# Autodesk Inventor assembly: stage1-planetary
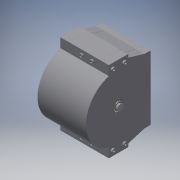
[picture p0: Inventor's stored thumbnail of the model, 180x180]
Saved by Autodesk Inventor 2019 (Build 230136000, 136)
## iProperties
Created: 2019-12-31
Part Number: stage1-planetary
Material: 一般
Document SubType Name: Assembly
Designer: user
Author: user
## Documents named in this file (23)
- D:\大學\大三上\機械設計(宋震國\stage1-planetary.iam
- D:\大學\大三上\機械設計(宋震國\Stage1\Gear_Housing_Bottom.ipt
- D:\大學\大三上\機械設計(宋震國\Stage1\carrier1.ipt
- D:\大學\大三上\機械設計(宋震國\Stage1\planet1.ipt
- D:\大學\大三上\機械設計(宋震國\Stage1\ring1.ipt
- D:\大學\大三上\機械設計(宋震國\Stage1\sun1.ipt
- D:\大學\大三上\機械設計(宋震國\stage1-planetary\機械便覽魔法師\軸5.iam
- D:\大學\大三上\機械設計(宋震國\stage1-planetary\機械便覽魔法師\軸承14.iam
- D:\大學\大三上\機械設計(宋震國\Stage1\planet2.ipt
- D:\大學\大三上\機械設計(宋震國\Stage1\ring2.ipt
- D:\大學\大三上\機械設計(宋震國\Stage1\sun2.ipt
- D:\大學\大三上\機械設計(宋震國\子彧-20200102T093658Z-001\子彧\最後確定\carrier2.ipt
- D:\大學\大三上\機械設計(宋震國\Stage1\Gear_Housing_Input_lid.ipt
- D:\大學\大三上\機械設計(宋震國\Stage1\Gear_Housing_Output_lid.ipt
- D:\大學\大三上\機械設計(宋震國\stage1-planetary\機械便覽魔法師\軸承15.iam
- D:\大學\大三上\機械設計(宋震國\stage1-planetary\機械便覽魔法師\軸承16.iam
- D:\大學\大三上\機械設計(宋震國\stage1-planetary\機械便覽魔法師\軸承17.iam
- D:\大學\大三上\機械設計(宋震國\stage1-planetary\機械便覽魔法師\軸承18.iam
- D:\大學\大三上\機械設計(宋震國\stage1-planetary\機械便覽魔法師\軸6.iam
- D:\大學\大三上\機械設計(宋震國\stage1-planetary\機械便覽魔法師\軸7.iam
- D:\大學\大三上\機械設計(宋震國\Stage1\Gear_Housing_Top2.ipt
- D:\大學\大三上\機械設計(宋震國\Stage1\M4set_screw.ipt
- D:\大學\大三上\機械設計(宋震國\Stage1\M6screw.ipt
## Components (69 placed, 12 different names)
1. Gear_Housing_Bottom:1 — 貼合:92, 貼合:93, 貼合:94, 貼合:95, 貼合:133, 貼合:134, 齊平:38, 貼合:143, 齊平:39, 齊平:41, 貼合:147, 齊平:42, 貼合:148
2. carrier1:1 — 貼合:74, 貼合:75, 貼合:76, 貼合:77, 貼合:78, 貼合:79, 貼合:80, 齊平:15, 齊平:16, 齊平:17, 貼合:176, 貼合:178, 貼合:179, 貼合:180, 貼合:181, 貼合:182, 貼合:183, 貼合:184, 貼合:185, 貼合:186, 貼合:187, 貼合:188, 貼合:189, 貼合:190, 貼合:191, 貼合:192
3. 正齒輪1:6 — 貼合:75, 貼合:84, 插入:2, 貼合:88, 齊平:20
4. 正齒輪2:1 — 貼合:73, 齊平:14, 齊平:21, 貼合:92, 貼合:93
5. 正齒輪1:7 — 貼合:73, 齊平:14, 貼合:74, 旋轉:1, 插入:5, 貼合:175, 貼合:197, 貼合:198
6. 軸:2 [sub-assembly] — 貼合:80, 齊平:17, 貼合:84
7. 正齒輪1:8 — 貼合:76, 貼合:81, 貼合:82, 貼合:87, 齊平:19, 齊平:21
8. 正齒輪1:9 — 貼合:77, 貼合:83, 貼合:85, 齊平:18, 旋轉:1
9. 軸:3 [sub-assembly] — 貼合:78, 齊平:15, 貼合:83, 貼合:86, 插入:4
10. 軸:4 [sub-assembly] — 貼合:79, 貼合:81, 齊平:16, 貼合:82, 插入:3
11. 軸承:1 [sub-assembly] — 貼合:85, 貼合:86, 齊平:18
12. 軸承:3 [sub-assembly] — 插入:3
13. 軸承:4 [sub-assembly] — 貼合:87, 齊平:19
14. 軸承:5 [sub-assembly] — 貼合:88, 齊平:20
15. 軸承:6 [sub-assembly] — 插入:4
16. 軸承:7 [sub-assembly] — 插入:2
17. 軸承:8 [sub-assembly] — 貼合:102, 齊平:28
18. 正齒輪1:11 — 貼合:94, 貼合:95, 貼合:96, 齊平:22, 齊平:36
19. 正齒輪1:12 — 貼合:102, 齊平:28, 貼合:105, 齊平:29, 貼合:106
20. 正齒輪1:13 — 貼合:96, 齊平:22, 貼合:124, 貼合:193, 貼合:194, 貼合:195, 貼合:196
21. 正齒輪1:15 — 貼合:103, 齊平:25, 齊平:32, 貼合:110, 貼合:113, 齊平:36
22. 軸:6 [sub-assembly] — 貼合:113, 貼合:117, 齊平:35, 貼合:119
23. 軸:7 [sub-assembly] — 貼合:116, 齊平:34, 貼合:122, 貼合:123
24. 軸:8 [sub-assembly] — 貼合:106, 貼合:107, 貼合:118, 齊平:33
25. 軸承:9 [sub-assembly] — 貼合:105, 齊平:29, 貼合:107
26. 軸承:12 [sub-assembly] — 齊平:32, 貼合:110, 貼合:119
27. 軸承:13 [sub-assembly] — 貼合:103, 齊平:25
28. 軸承:14 [sub-assembly] — 貼合:120, 貼合:121, 貼合:122
29. carrier2:1 — 貼合:116, 貼合:117, 貼合:118, 齊平:33, 齊平:34, 齊平:35, 貼合:124, 貼合:145, 貼合:199, 貼合:200, 貼合:201, 貼合:202, 貼合:203, 貼合:204
30. 正齒輪1:16 — 貼合:120, 貼合:121, 貼合:123
31. Gear_Housing_Input_lid:1 — 貼合:135, 貼合:136, 貼合:137, 貼合:138, 齊平:38, 貼合:143, 貼合:153, 貼合:160, 貼合:161, 貼合:162, 貼合:163, 貼合:164, 貼合:165, 貼合:166
32. Gear_Housing_Output_lid:1 — 貼合:139, 貼合:140, 貼合:141, 齊平:37, 齊平:39, 貼合:148, 貼合:149, 貼合:167, 貼合:168, 貼合:169, 貼合:170, 貼合:171, 貼合:172, 貼合:173, 貼合:174
33. 軸承:15 [sub-assembly] — 貼合:135, 貼合:136
34. 軸承:16 [sub-assembly] — 貼合:137, 貼合:138, 貼合:142
35. 軸承:17 [sub-assembly] — 貼合:139, 貼合:140
36. 軸承:18 [sub-assembly] — 貼合:141, 齊平:37, 插入:6
37. 軸:11 [sub-assembly] — 貼合:145, 插入:6
38. 軸:12 [sub-assembly] — 插入:5, 貼合:142
39. Gear_Housing_Top2:1 — 貼合:147, 齊平:42, 貼合:149, 貼合:151, 貼合:152, 貼合:154, 貼合:155, 貼合:156, 貼合:157, 貼合:158, 貼合:159
40. M4set_screw:1 — 貼合:179, 貼合:180
41. M6screw:1 — 貼合:151, 貼合:159
42. M4set_screw:2 — 貼合:176, 貼合:182
43. M6screw:2 — 貼合:152, 貼合:158
44. M4set_screw:3 — 貼合:178, 貼合:181
45. M6screw:3 — 貼合:153, 貼合:160
46. M4set_screw:4 — 貼合:175
47. M6screw:4 — 貼合:167, 貼合:171
48. M4set_screw:5 — 貼合:183, 貼合:184
49. M6screw:5 — 貼合:156, 貼合:157
50. M4set_screw:6 — 貼合:187, 貼合:188
51. M6screw:6 — 貼合:154, 貼合:155
52. M6screw:7 — 貼合:168, 貼合:174
53. M6screw:8 — 貼合:161, 貼合:162
54. M6screw:9 — 貼合:163, 貼合:164
55. M6screw:10 — 貼合:165, 貼合:166
56. M6screw:11 — 貼合:170, 貼合:172
57. M6screw:12 — 貼合:169, 貼合:173
58. M4set_screw:7
59. M4set_screw:8 — 貼合:185, 貼合:186
60. M4set_screw:9
61. M4set_screw:10
62. M4set_screw:11 — 貼合:189, 貼合:190
63. M4set_screw:12 — 貼合:191, 貼合:192
64. M4set_screw:13 — 貼合:193, 貼合:195
65. M4set_screw:14 — 貼合:194, 貼合:196
66. M4set_screw:15 — 貼合:197, 貼合:198
67. M4set_screw:16 — 貼合:203, 貼合:204
68. M4set_screw:18 — 貼合:201, 貼合:202
69. M4set_screw:19 — 貼合:199, 貼合:200
## Relationships (134: Mate 105, Flush 22, Insert 5, Angle 1, RelateRotation 1)
- 角度:1 [Angle] (0 deg)
- 貼合:73 [Mate]: 正齒輪2:1 ↔ 正齒輪1:7
- 齊平:14 [Flush]: 正齒輪2:1 ↔ 正齒輪1:7
- 貼合:74 [Mate]: carrier1:1 ↔ 正齒輪1:7
- 貼合:75 [Mate]: carrier1:1 ↔ 正齒輪1:6
- 貼合:76 [Mate]: carrier1:1 ↔ 正齒輪1:8
- 貼合:77 [Mate]: carrier1:1 ↔ 正齒輪1:9
- 貼合:78 [Mate]: carrier1:1 ↔ 軸:3
- 貼合:79 [Mate]: carrier1:1 ↔ 軸:4
- 貼合:80 [Mate]: carrier1:1 ↔ 軸:2
- 貼合:81 [Mate]: 正齒輪1:8 ↔ 軸:4
- 齊平:15 [Flush]: carrier1:1 ↔ 軸:3
- 齊平:16 [Flush]: carrier1:1 ↔ 軸:4
- 齊平:17 [Flush]: carrier1:1 ↔ 軸:2
- 貼合:82 [Mate]: 正齒輪1:8 ↔ 軸:4
- 貼合:83 [Mate]: 正齒輪1:9 ↔ 軸:3
- 貼合:84 [Mate]: 正齒輪1:6 ↔ 軸:2
- 貼合:85 [Mate]: 正齒輪1:9 ↔ 軸承:1
- 貼合:86 [Mate]: 軸:3 ↔ 軸承:1
- 齊平:18 [Flush]: 正齒輪1:9 ↔ 軸承:1
- 貼合:87 [Mate]: 正齒輪1:8 ↔ 軸承:4
- 齊平:19 [Flush]: 正齒輪1:8 ↔ 軸承:4
- 插入:2 [Insert]: 正齒輪1:6 ↔ 軸承:7
- 貼合:88 [Mate]: 正齒輪1:6 ↔ 軸承:5
- 齊平:20 [Flush]: 正齒輪1:6 ↔ 軸承:5
- 插入:3 [Insert]: 軸:4 ↔ 軸承:3
- 插入:4 [Insert]: 軸:3 ↔ 軸承:6
- 齊平:21 [Flush]: 正齒輪2:1 ↔ 正齒輪1:8
- 旋轉:1 [RelateRotation] (1 ul): 正齒輪1:7 ↔ 正齒輪1:9
- 貼合:92 [Mate]: Gear_Housing_Bottom:1 ↔ 正齒輪2:1
- 貼合:93 [Mate]: Gear_Housing_Bottom:1 ↔ 正齒輪2:1
- 貼合:94 [Mate]: Gear_Housing_Bottom:1 ↔ 正齒輪1:11
- 貼合:95 [Mate]: Gear_Housing_Bottom:1 ↔ 正齒輪1:11
- 貼合:96 [Mate]: 正齒輪1:11 ↔ 正齒輪1:13
- 齊平:22 [Flush]: 正齒輪1:11 ↔ 正齒輪1:13
- 貼合:102 [Mate]: 軸承:8 ↔ 正齒輪1:12
- 貼合:103 [Mate]: 正齒輪1:15 ↔ 軸承:13
- 齊平:25 [Flush]: 正齒輪1:15 ↔ 軸承:13
- 齊平:28 [Flush]: 軸承:8 ↔ 正齒輪1:12
- 貼合:105 [Mate]: 正齒輪1:12 ↔ 軸承:9
- 齊平:29 [Flush]: 正齒輪1:12 ↔ 軸承:9
- 貼合:106 [Mate]: 正齒輪1:12 ↔ 軸:8
- 貼合:107 [Mate]: 軸:8 ↔ 軸承:9
- 齊平:32 [Flush]: 正齒輪1:15 ↔ 軸承:12
- 貼合:110 [Mate]: 正齒輪1:15 ↔ 軸承:12
- 貼合:113 [Mate]: 正齒輪1:15 ↔ 軸:6
- 貼合:116 [Mate]: 軸:7 ↔ carrier2:1
- 貼合:117 [Mate]: 軸:6 ↔ carrier2:1
- 貼合:118 [Mate]: 軸:8 ↔ carrier2:1
- 齊平:33 [Flush]: 軸:8 ↔ carrier2:1
- 齊平:34 [Flush]: 軸:7 ↔ carrier2:1
- 齊平:35 [Flush]: 軸:6 ↔ carrier2:1
- 貼合:119 [Mate]: 軸:6 ↔ 軸承:12
- 貼合:120 [Mate]: 軸承:14 ↔ 正齒輪1:16
- 貼合:121 [Mate]: 軸承:14 ↔ 正齒輪1:16
- 貼合:122 [Mate]: 軸:7 ↔ 軸承:14
- 貼合:123 [Mate]: 軸:7 ↔ 正齒輪1:16
- 齊平:36 [Flush]: 正齒輪1:11 ↔ 正齒輪1:15
- 貼合:124 [Mate]: 正齒輪1:13 ↔ carrier2:1
- 貼合:133 [Mate]: Gear_Housing_Bottom:1
- 貼合:134 [Mate]: Gear_Housing_Bottom:1
- 貼合:135 [Mate]: Gear_Housing_Input_lid:1 ↔ 軸承:15
- 貼合:136 [Mate]: Gear_Housing_Input_lid:1 ↔ 軸承:15
- 貼合:137 [Mate]: Gear_Housing_Input_lid:1 ↔ 軸承:16
- 貼合:138 [Mate]: Gear_Housing_Input_lid:1 ↔ 軸承:16
- 貼合:139 [Mate]: Gear_Housing_Output_lid:1 ↔ 軸承:17
- 貼合:140 [Mate]: Gear_Housing_Output_lid:1 ↔ 軸承:17
- 貼合:141 [Mate]: Gear_Housing_Output_lid:1 ↔ 軸承:18
- 齊平:37 [Flush]: Gear_Housing_Output_lid:1 ↔ 軸承:18
- 插入:5 [Insert]: 正齒輪1:7 ↔ 軸:12
- 貼合:142 [Mate]: 軸承:16 ↔ 軸:12
- 齊平:38 [Flush]: Gear_Housing_Bottom:1 ↔ Gear_Housing_Input_lid:1
- 貼合:143 [Mate]: Gear_Housing_Bottom:1 ↔ Gear_Housing_Input_lid:1
- 貼合:145 [Mate]: carrier2:1 ↔ 軸:11
- 齊平:39 [Flush]: Gear_Housing_Bottom:1 ↔ Gear_Housing_Output_lid:1
- 插入:6 [Insert]: 軸承:18 ↔ 軸:11
- 齊平:41 [Flush]: Gear_Housing_Bottom:1
- 貼合:147 [Mate]: Gear_Housing_Bottom:1 ↔ Gear_Housing_Top2:1
- 齊平:42 [Flush]: Gear_Housing_Bottom:1 ↔ Gear_Housing_Top2:1
- 貼合:148 [Mate]: Gear_Housing_Bottom:1 ↔ Gear_Housing_Output_lid:1
- 貼合:149 [Mate]: Gear_Housing_Output_lid:1 ↔ Gear_Housing_Top2:1
- 貼合:151 [Mate]: Gear_Housing_Top2:1 ↔ M6screw:1
- 貼合:152 [Mate]: Gear_Housing_Top2:1 ↔ M6screw:2
- 貼合:153 [Mate]: Gear_Housing_Input_lid:1 ↔ M6screw:3
- 貼合:154 [Mate]: Gear_Housing_Top2:1 ↔ M6screw:6
- 貼合:155 [Mate]: Gear_Housing_Top2:1 ↔ M6screw:6
- 貼合:156 [Mate]: Gear_Housing_Top2:1 ↔ M6screw:5
- 貼合:157 [Mate]: Gear_Housing_Top2:1 ↔ M6screw:5
- 貼合:158 [Mate]: Gear_Housing_Top2:1 ↔ M6screw:2
- 貼合:159 [Mate]: Gear_Housing_Top2:1 ↔ M6screw:1
- 貼合:160 [Mate]: Gear_Housing_Input_lid:1 ↔ M6screw:3
- 貼合:161 [Mate]: Gear_Housing_Input_lid:1 ↔ M6screw:8
- 貼合:162 [Mate]: Gear_Housing_Input_lid:1 ↔ M6screw:8
- 貼合:163 [Mate]: Gear_Housing_Input_lid:1 ↔ M6screw:9
- 貼合:164 [Mate]: Gear_Housing_Input_lid:1 ↔ M6screw:9
- 貼合:165 [Mate]: Gear_Housing_Input_lid:1 ↔ M6screw:10
- 貼合:166 [Mate]: Gear_Housing_Input_lid:1 ↔ M6screw:10
- 貼合:167 [Mate]: Gear_Housing_Output_lid:1 ↔ M6screw:4
- 貼合:168 [Mate]: Gear_Housing_Output_lid:1 ↔ M6screw:7
- 貼合:169 [Mate]: Gear_Housing_Output_lid:1 ↔ M6screw:12
- 貼合:170 [Mate]: Gear_Housing_Output_lid:1 ↔ M6screw:11
- 貼合:171 [Mate]: Gear_Housing_Output_lid:1 ↔ M6screw:4
- 貼合:172 [Mate]: Gear_Housing_Output_lid:1 ↔ M6screw:11
- 貼合:173 [Mate]: Gear_Housing_Output_lid:1 ↔ M6screw:12
- 貼合:174 [Mate]: Gear_Housing_Output_lid:1 ↔ M6screw:7
- 貼合:175 [Mate]: 正齒輪1:7 ↔ M4set_screw:4
- 貼合:176 [Mate]: carrier1:1 ↔ M4set_screw:2
- 貼合:178 [Mate]: carrier1:1 ↔ M4set_screw:3
- 貼合:179 [Mate]: carrier1:1 ↔ M4set_screw:1
- 貼合:180 [Mate] (-16 mm): carrier1:1 ↔ M4set_screw:1
- 貼合:181 [Mate] (-14.5 mm): carrier1:1 ↔ M4set_screw:3
- 貼合:182 [Mate] (-15 mm): carrier1:1 ↔ M4set_screw:2
- 貼合:183 [Mate]: carrier1:1 ↔ M4set_screw:5
- 貼合:184 [Mate] (-15 mm): carrier1:1 ↔ M4set_screw:5
- 貼合:185 [Mate]: carrier1:1 ↔ M4set_screw:8
- 貼合:186 [Mate] (-15 mm): carrier1:1 ↔ M4set_screw:8
- 貼合:187 [Mate]: carrier1:1 ↔ M4set_screw:6
- 貼合:188 [Mate] (-15 mm): carrier1:1 ↔ M4set_screw:6
- 貼合:189 [Mate]: carrier1:1 ↔ M4set_screw:11
- 貼合:190 [Mate] (-15 mm): carrier1:1 ↔ M4set_screw:11
- 貼合:191 [Mate]: carrier1:1 ↔ M4set_screw:12
- 貼合:192 [Mate] (-15 mm): carrier1:1 ↔ M4set_screw:12
- 貼合:193 [Mate]: 正齒輪1:13 ↔ M4set_screw:13
- 貼合:194 [Mate]: 正齒輪1:13 ↔ M4set_screw:14
- 貼合:195 [Mate] (-15 mm): 正齒輪1:13 ↔ M4set_screw:13
- 貼合:196 [Mate] (-15 mm): 正齒輪1:13 ↔ M4set_screw:14
- 貼合:197 [Mate]: 正齒輪1:7 ↔ M4set_screw:15
- 貼合:198 [Mate] (-22 mm): 正齒輪1:7 ↔ M4set_screw:15
- 貼合:199 [Mate]: carrier2:1 ↔ M4set_screw:19
- 貼合:200 [Mate] (-15 mm): carrier2:1 ↔ M4set_screw:19
- 貼合:201 [Mate]: carrier2:1 ↔ M4set_screw:18
- 貼合:202 [Mate] (-15 mm): carrier2:1 ↔ M4set_screw:18
- 貼合:203 [Mate]: carrier2:1 ↔ M4set_screw:16
- 貼合:204 [Mate] (-15 mm): carrier2:1 ↔ M4set_screw:16
